# Autodesk Inventor assembly: 4in Lazy Suzan
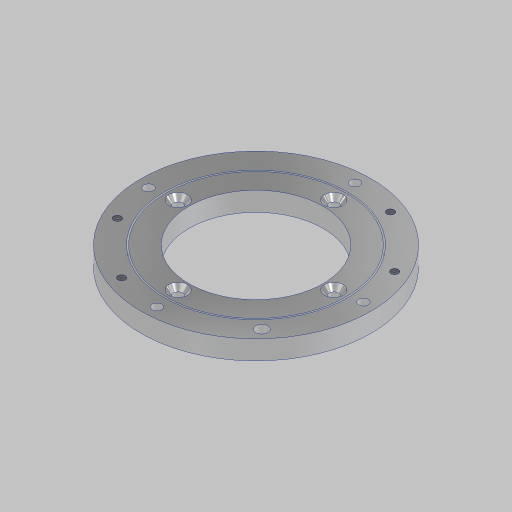
[picture p0: Inventor's stored thumbnail of the model, 512x512]
Saved by Autodesk Inventor 2023.5 (Build 275446000, 446)
## iProperties
Created: 2025-02-23
Part Number: 4in Lazy Suzan
Document SubType Name: Assembly
Designer: brand
Catalog Web Link: https://www.amazon.com/Aluminium-Turntable-Bearing-Rotating-Hardware/dp/B08CSMYXFV/ref=sr_1_4_sspa?dib=eyJ2IjoiMSJ9._dIJFbhkyI92XmDmKNkxFgU_0ePHUSC9YqSv3sFBVjlsdRyExycsbXiQU_MUmMUvJGy9GCAPT9QtxClaBTku0FbfhZoCtIpOYngGBTnJo919GddPBDS83ooZRsxJG5R7jq3cNUDygyRS_OmJipfkoM5OCq8T20qhxkRWpoecfTOp-jOGMSp8e54UpLORAgNJtiqEyScbtuTVsJE3J9O2aar2usHcvoaSkqYkZJUQvearKUFKK2c7Wpxg1pH32h2YCQUZluVIHso0mULp-QWUF_UNj0rclYvDnB-_XJVLeZI.44kslggF-zdLCPfpDMEyn6Enj3QOh1QtcF3QqGoJ9Ac&dib_tag=se&keywords=mini%2Blazy%2Bsusan&qid=1740338553&sr=8-4-spons&sp_csd=d2lkZ2V0TmFtZT1zcF9hdGY&th=1
Author: brand
## Documents named in this file (3)
- C:\Users\slick\OneDrive\Desktop\2025-ReefScape---CAD\COMMON PARTS\4in Lazy Suzan.iam
- C:\Users\slick\OneDrive\Desktop\2025-ReefScape---CAD\COMMON PARTS\4in LS-001.ipt
- C:\Users\slick\OneDrive\Desktop\2025-ReefScape---CAD\COMMON PARTS\4in LS-002.ipt
## Components (2 placed, 2 different names)
1. 4in LS-001:1 — Insert:1
2. 4in LS-002:1 — Insert:1
## Relationships (1: Insert 1)
- Insert:1: 4in LS-001:1 ↔ 4in LS-002:1
